# Autodesk Inventor assembly: carromrobot
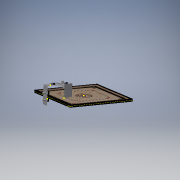
[picture p0: Inventor's stored thumbnail of the model, 180x180]
Saved by Autodesk Inventor 2019 (Build 230136000, 136)
## iProperties
Created: 2020-03-03
Part Number: carromrobot
Document SubType Name: Assembly
Designer: Dell
Author: Dell
## Documents named in this file (3)
- C:\Users\Dell\Documents\carromrobot.iam
- C:\Users\Dell\Downloads\carrom board.ipt
- C:\Users\Dell\Documents\finalassembly.iam
## Components (2 placed, 2 different names)
1. carrom board:1 — Rigid:1
2. finalassembly:1 [sub-assembly] — Rigid:1
## Relationships (1: WeldJoint 1)
- Rigid:1 [WeldJoint]: carrom board:1 ↔ finalassembly:1
